# Autodesk Inventor assembly: Корпус
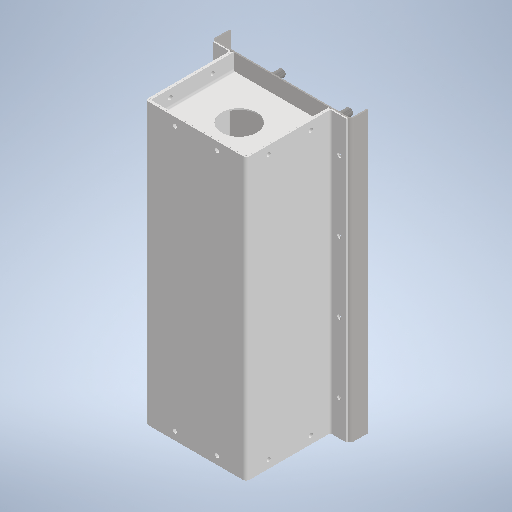
[picture p0: Inventor's stored thumbnail of the model, 512x512]
Saved by Autodesk Inventor 2025 (Build 290162010, 162A)
## iProperties
Created: 2024-04-16
Part Number: Корпус
Document SubType Name: Assembly
Designer: pokla
Author: pokla
## Documents named in this file (6)
- C:\Users\pokla\Documents\Inventor\Gusev_Meshalka\ASY Мешалка\Корпус.iam
- C:\Users\pokla\Documents\Inventor\Gusev_Meshalka\ASY Мешалка\Крепление.ipt
- C:\Users\pokla\Documents\Inventor\Gusev_Meshalka\ASY Мешалка\Крепление корпуса.ipt
- C:\Users\pokla\Documents\Inventor\Gusev_Meshalka\ASY Мешалка\Параметры.ipt
- C:\Users\pokla\Documents\Inventor\Gusev_Meshalka\ASY Мешалка\Кожух.ipt
- C:\Users\pokla\Documents\Inventor\Content Center Files\R2025\en-US\CSN EN 24015\CSN EN 24015 - M10x50.ipt
## Components (9 placed, 5 different names)
1. Крепление.ipt:1 — Flush:1, Mate:1, Rigid:7, Rigid:8, Insert:1
2. Параметры.ipt:1
3. Кожух.ipt:1 — Rigid:9
4. Крепление корпуса.ipt:1 — Rigid:7, Rigid:9
5. Крепление корпуса.ipt:2 — Rigid:8
6. CSN EN 24015 - M10x50.ipt:1 — Insert:1
7. CSN EN 24015 - M10x50.ipt:2
8. CSN EN 24015 - M10x50.ipt:3
9. CSN EN 24015 - M10x50.ipt:4
## Component patterns: (4 elements, first: CSN EN 24015 - M10x50.ipt:1)
## Relationships (6: WeldJoint 3, Flush 1, Mate 1, Insert 1)
- Flush:1: Крепление.ipt:1
- Mate:1: Крепление.ipt:1
- Rigid:7 [WeldJoint] (-23 mm): Крепление.ipt:1 ↔ Крепление корпуса.ipt:1
- Rigid:8 [WeldJoint] (-23 mm): Крепление.ipt:1 ↔ Крепление корпуса.ipt:2
- Rigid:9 [WeldJoint]: Кожух.ipt:1 ↔ Крепление корпуса.ipt:1
- Insert:1: Крепление.ipt:1 ↔ CSN EN 24015 - M10x50.ipt:1
